# Autodesk Inventor assembly: 276-2243
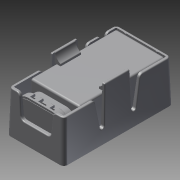
[picture p0: Inventor's stored thumbnail of the model, 180x180]
Saved by Autodesk Inventor 2013 (Build 170138000, 138)
## iProperties
Category: Power
Company: Autodesk Inc.
Created: 2012-02-07
Part Number: 276-2243
Document SubType Name: Assembly
Designer: Autodesk Inc.
Catalog Web Link: http://www.vexrobotics.com/276-2243.html
Description: VEXnet Backup Battery Holder
Vendor: VEX
Author: Autodesk Inc.
## Documents named in this file (5)
- C:\Data Folder\VEX 2012\VEX KOP Uploads\2013\Imperial\Power\VEXnet Backup Battery Holder.iam
- C:\Data Folder\VEX 2012\VEX KOP Uploads\2013\Imperial\Power\Components\9V-BATTERY.ipt
- C:\Data Folder\VEX 2012\VEX KOP Uploads\2013\Imperial\Power\Components\BATTERY-HOLDER.ipt
- C:\Data Folder\VEX 2012\VEX KOP Uploads\2013\Imperial\Power\Components\CONTACT-BACK-CAP.ipt
- C:\Data Folder\VEX 2012\VEX KOP Uploads\2013\Imperial\Power\Components\CONTACT-INSULATOR-CAP.ipt
## Components (4 placed, 4 different names)
1. BATTERY-HOLDER:1 — Mate:1, Mate:2, Mate:3
2. 9V-BATTERY:1 — Mate:1, Mate:2, Mate:3, Mate:7, Mate:8, Mate:9
3. CONTACT-BACK-CAP:1 — Flush:1, Mate:10, Mate:11
4. CONTACT-INSULATOR-CAP:1 — Mate:7, Mate:8, Mate:9, Flush:1, Mate:10, Mate:11
## Relationships (9: Mate 8, Flush 1)
- Mate:1: BATTERY-HOLDER:1 ↔ 9V-BATTERY:1
- Mate:2: BATTERY-HOLDER:1 ↔ 9V-BATTERY:1
- Mate:3: BATTERY-HOLDER:1 ↔ 9V-BATTERY:1
- Mate:7: 9V-BATTERY:1 ↔ CONTACT-INSULATOR-CAP:1
- Mate:8: 9V-BATTERY:1 ↔ CONTACT-INSULATOR-CAP:1
- Mate:9: 9V-BATTERY:1 ↔ CONTACT-INSULATOR-CAP:1
- Flush:1: CONTACT-BACK-CAP:1 ↔ CONTACT-INSULATOR-CAP:1
- Mate:10: CONTACT-BACK-CAP:1 ↔ CONTACT-INSULATOR-CAP:1
- Mate:11: CONTACT-BACK-CAP:1 ↔ CONTACT-INSULATOR-CAP:1
